# Autodesk Inventor assembly: 870-00687 Assembly Tray Cargo
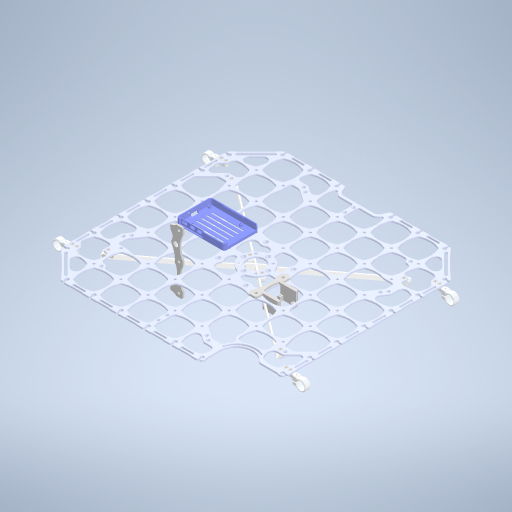
[picture p0: Inventor's stored thumbnail of the model, 512x512]
Saved by Autodesk Inventor 2024 (Build 280153000, 153)
## iProperties
Created: 2021-03-30
Part Number: 870-00687 Assembly Tray Cargo
Description: STEP AP214
Document SubType Name: Assembly
Designer: Eli
Title: 870-00687 Assembly Tray Cargo.STEP
Revision Number: ANY
Sending System: SolidWorks 2020
Preprocessor: SwSTEP 2.0
## Documents named in this file (11)
- C:\Users\Eli\Documents\GitHub\3D-design\Alta X\870-00687 Assembly Tray Cargo\870-00687 Assembly Tray Cargo.iam
- C:\Users\Eli\Documents\GitHub\3D-design\Alta X\870-00687 Assembly Tray Cargo\445-00217 Tray Cargo.ipt
- C:\Users\Eli\Documents\GitHub\3D-design\Alta X\870-00687 Assembly Tray Cargo\470-00297 Bolt M3 x 8 FHCS Dacromet_91294A128.ipt
- C:\Users\Eli\Documents\GitHub\3D-design\Alta X\870-00687 Assembly Tray Cargo\445-00218 Stiffener Tray Cargo.ipt
- C:\Users\Eli\Documents\GitHub\3D-design\Alta X\870-00687 Assembly Tray Cargo\410-00966 Clamp 15mm Accessory Mount.ipt
- C:\Users\Eli\Documents\GitHub\3D-design\Alta X\870-00687 Assembly Tray Cargo\410-00914 Angled Block M3_M3.ipt
- C:\Users\Eli\Documents\GitHub\3D-design\Alta X\870-00687 Assembly Tray Cargo\470-00294 Bolt M3 x 10 SHCS Dacromet_95263A134.ipt
- C:\Users\Eli\Documents\GitHub\3D-design\Alta X\Bottom.ipt
- C:\Users\Eli\Documents\GitHub\3D-design\Alta X\lepton mount.ipt
- C:\Users\Eli\Documents\GitHub\3D-design\Alta X\alta plate for lepton.ipt
- C:\Users\Eli\Documents\GitHub\3D-design\Alta X\alta plate razz pi.ipt
## Components (47 placed, 47 different names)
1. 445-00217 Tray Cargo_1 — Insert:1, Insert:2
2. 470-00297 Bolt M3 x 8 FHCS Dacromet_91294A128_2
3. 470-00297 Bolt M3 x 8 FHCS Dacromet_91294A128_3
4. 470-00297 Bolt M3 x 8 FHCS Dacromet_91294A128_4
5. 470-00297 Bolt M3 x 8 FHCS Dacromet_91294A128_5
6. 470-00297 Bolt M3 x 8 FHCS Dacromet_91294A128_6
7. 470-00297 Bolt M3 x 8 FHCS Dacromet_91294A128_7
8. 470-00297 Bolt M3 x 8 FHCS Dacromet_91294A128_8
9. 470-00297 Bolt M3 x 8 FHCS Dacromet_91294A128_9
10. 470-00297 Bolt M3 x 8 FHCS Dacromet_91294A128_10
11. 470-00297 Bolt M3 x 8 FHCS Dacromet_91294A128_11
12. 470-00297 Bolt M3 x 8 FHCS Dacromet_91294A128_12
13. 470-00297 Bolt M3 x 8 FHCS Dacromet_91294A128_13
14. 470-00297 Bolt M3 x 8 FHCS Dacromet_91294A128_14
15. 470-00297 Bolt M3 x 8 FHCS Dacromet_91294A128_15
16. 445-00218 Stiffener Tray Cargo_16
17. 445-00218 Stiffener Tray Cargo_17
18. 410-00966 Clamp 15mm Accessory Mount_18
19. 410-00966 Clamp 15mm Accessory Mount_19
20. 410-00966 Clamp 15mm Accessory Mount_20
21. 410-00966 Clamp 15mm Accessory Mount_21
22. 410-00914 Angled Block M3_M3_22
23. 410-00914 Angled Block M3_M3_23
24. 410-00914 Angled Block M3_M3_24
25. 410-00914 Angled Block M3_M3_25
26. 410-00914 Angled Block M3_M3_26
27. 410-00914 Angled Block M3_M3_27
28. 470-00297 Bolt M3 x 8 FHCS Dacromet_91294A128_28
29. 470-00297 Bolt M3 x 8 FHCS Dacromet_91294A128_29
30. 470-00297 Bolt M3 x 8 FHCS Dacromet_91294A128_30
31. 470-00297 Bolt M3 x 8 FHCS Dacromet_91294A128_31
32. 470-00297 Bolt M3 x 8 FHCS Dacromet_91294A128_32
33. 470-00297 Bolt M3 x 8 FHCS Dacromet_91294A128_33
34. 470-00297 Bolt M3 x 8 FHCS Dacromet_91294A128_34
35. 470-00297 Bolt M3 x 8 FHCS Dacromet_91294A128_35
36. 470-00297 Bolt M3 x 8 FHCS Dacromet_91294A128_36
37. 470-00297 Bolt M3 x 8 FHCS Dacromet_91294A128_37
38. 470-00297 Bolt M3 x 8 FHCS Dacromet_91294A128_38
39. 470-00297 Bolt M3 x 8 FHCS Dacromet_91294A128_39
40. 470-00294 Bolt M3 x 10 SHCS Dacromet_95263A134_40
41. 470-00294 Bolt M3 x 10 SHCS Dacromet_95263A134_41
42. 470-00294 Bolt M3 x 10 SHCS Dacromet_95263A134_42
43. 470-00294 Bolt M3 x 10 SHCS Dacromet_95263A134_43
44. Bottom:1
45. lepton mount:1 — Flush:1
46. alta plate for lepton:1 — Insert:1, Insert:2, Flush:1
47. alta plate razz pi:1
## Relationships (3: Insert 2, Flush 1)
- Insert:1: 445-00217 Tray Cargo_1 ↔ alta plate for lepton:1
- Insert:2: 445-00217 Tray Cargo_1 ↔ alta plate for lepton:1
- Flush:1: lepton mount:1 ↔ alta plate for lepton:1
